# Autodesk Inventor assembly: Assembly_All_V02
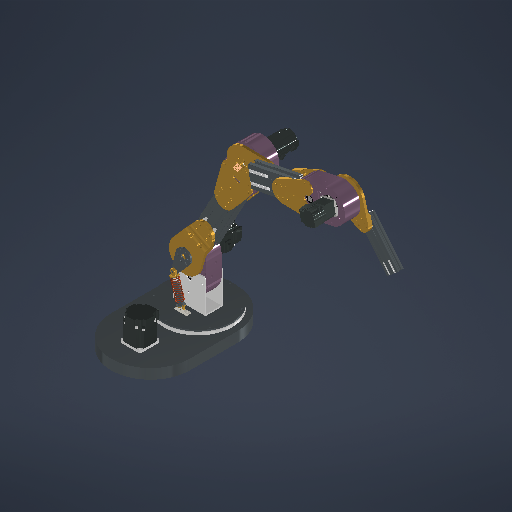
[picture p0: Inventor's stored thumbnail of the model, 512x512]
Saved by Autodesk Inventor 2026 (Build 300175000, 175)
## iProperties
Created: 2025-12-01
Part Number: Assembly_All_V02
Document SubType Name: Assembly
Designer: DanielFGarzon
Mass: 8745.83 g
Surface Area: 15813.7 cm^2
Volume: 3977 cm^3
Author: DanielFGarzon
## Documents named in this file (11)
- D:\POLIMI\3RD SEMESTER\Industrial Robotics\Project\Mine\Assembly_All_V03.iam
- D:\POLIMI\3RD SEMESTER\Industrial Robotics\Project\Mine\Base_Assembly_V02.iam
- D:\POLIMI\3RD SEMESTER\Industrial Robotics\Project\Mine\Link_00_Assembly_V02.iam
- D:\POLIMI\3RD SEMESTER\Industrial Robotics\Project\Mine\Bottom_Spring.ipt
- D:\POLIMI\3RD SEMESTER\Industrial Robotics\Project\Mine\Top_Spring.ipt
- D:\POLIMI\3RD SEMESTER\Industrial Robotics\Project\Mine\Counter_Balance_01.ipt
- D:\POLIMI\3RD SEMESTER\Industrial Robotics\Project\Mine\Counter_Balance_GND.ipt
- D:\POLIMI\3RD SEMESTER\Industrial Robotics\Project\Mine\Spring_Spring.ipt
- D:\POLIMI\3RD SEMESTER\Industrial Robotics\Project\Mine\Link_01_Assembly_V03.iam
- D:\POLIMI\3RD SEMESTER\Industrial Robotics\Project\Mine\Link_02_Assembly_V03.iam
- D:\POLIMI\3RD SEMESTER\Industrial Robotics\Project\Mine\Link_03_Assembly_V03.iam
## Components (10 placed, 10 different names)
1. Base_Assembly_V02:1 [sub-assembly] — Mate:2, Mate:3, Mate:7, Mate:8, Mate:9, Mate:10
2. Link_00_Assembly_V02:1 [sub-assembly] — Mate:2, Mate:3, Mate:19, Mate:20, Mate:21, Mate:38, Rotational:1
3. Link_01_Assembly_V03:1 [sub-assembly] — Mate:38, Rotational:1, Mate:41, Mate:42, Mate:43, Rotational:4
4. Link_02_Assembly_V03:1 [sub-assembly] — Rotational:3, Rotational:4
5. Link_03_Assembly_V03:1 [sub-assembly] — Rotational:3
6. Counter_Balance_01:1 — Mate:41, Mate:42, Mate:43, Mate:44
7. Counter_Balance_GND:1 — Mate:19, Mate:20, Mate:21, Mate:30, Mate:31
8. Bottom_Spring:1 — Mate:30, Mate:31, Mate:37, Mate:32, Mate:35, Mate:36
9. Top_Spring:1 — Mate:37, Mate:32, Mate:34, Mate:44
10. Spring_Spring:1 — Mate:34, Mate:35, Mate:36
## Relationships (24: Mate 21, RevoluteJoint 3)
- Mate:2: Base_Assembly_V02:1 ↔ Link_00_Assembly_V02:1
- Mate:3: Base_Assembly_V02:1 ↔ Link_00_Assembly_V02:1
- Mate:7: Base_Assembly_V02:1
- Mate:8: Base_Assembly_V02:1
- Mate:9: Base_Assembly_V02:1
- Mate:10: Base_Assembly_V02:1
- Mate:19: Link_00_Assembly_V02:1 ↔ Counter_Balance_GND:1
- Mate:20: Link_00_Assembly_V02:1 ↔ Counter_Balance_GND:1
- Mate:21: Link_00_Assembly_V02:1 ↔ Counter_Balance_GND:1
- Mate:30: Counter_Balance_GND:1 ↔ Bottom_Spring:1
- Mate:31: Counter_Balance_GND:1 ↔ Bottom_Spring:1
- Mate:37 (58 mm): Bottom_Spring:1 ↔ Top_Spring:1
- Mate:32: Bottom_Spring:1 ↔ Top_Spring:1
- Mate:34: Top_Spring:1 ↔ Spring_Spring:1
- Mate:35: Bottom_Spring:1 ↔ Spring_Spring:1
- Mate:36: Bottom_Spring:1 ↔ Spring_Spring:1
- Mate:38: Link_00_Assembly_V02:1 ↔ Link_01_Assembly_V03:1
- Rotational:1 [RevoluteJoint]: Link_00_Assembly_V02:1 ↔ Link_01_Assembly_V03:1
- Mate:41: Link_01_Assembly_V03:1 ↔ Counter_Balance_01:1
- Mate:42: Link_01_Assembly_V03:1 ↔ Counter_Balance_01:1
- Mate:43: Link_01_Assembly_V03:1 ↔ Counter_Balance_01:1
- Mate:44: Counter_Balance_01:1 ↔ Top_Spring:1
- Rotational:3 [RevoluteJoint]: Link_02_Assembly_V03:1 ↔ Link_03_Assembly_V03:1
- Rotational:4 [RevoluteJoint]: Link_01_Assembly_V03:1 ↔ Link_02_Assembly_V03:1
